# Autodesk Inventor assembly: Field plates
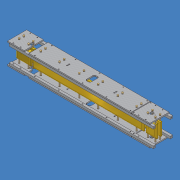
[picture p0: Inventor's stored thumbnail of the model, 180x180]
Saved by Autodesk Inventor 2011 (Build 150239000, 239)
## iProperties
Created: 2005-07-04
Part Number: Field plates
Document SubType Name: Assembly
Designer: jony
Author: jony
## Documents named in this file (5)
- C:\Users\Joe\Inventor\EDM Beamline 2010\EDM Beamline\Field plates\Field plates.iam
- C:\Users\Joe\Inventor\EDM Beamline 2010\EDM Beamline\Field plates\Plate support assembly.iam
- C:\Users\Joe\Inventor\EDM Beamline 2010\EDM Beamline\Field plates\Lower guard assembly.iam
- C:\Users\Joe\Inventor\EDM Beamline 2010\EDM Beamline\Field plates\Upper guard assembly.iam
- C:\Users\Joe\Inventor\EDM Beamline 2010\EDM Beamline\Field plates\C plate assembly.iam
## Components (8 placed, 4 different names)
1. Plate support assembly:1 [sub-assembly] — Mate:1, Mate:2, Mate:3, Mate:4, Mate:7, Mate:8, Mate:9, Mate:10, Mate:11, Mate:12, Mate:13, Mate:14, Mate:15, Mate:16, Mate:17, Mate:18, Mate:19, Mate:20, Mate:21
2. Plate support assembly:2 [sub-assembly] — Mate:5, Mate:6, Mate:15
3. Lower guard assembly:1 [sub-assembly] — Mate:1, Mate:2, Mate:5, Mate:6, Mate:16
4. Lower guard assembly:2 [sub-assembly] — Mate:3, Mate:4, Mate:17
5. Upper guard assembly:1 [sub-assembly] — Mate:7, Mate:8, Mate:18
6. Upper guard assembly:2 [sub-assembly] — Mate:9, Mate:10, Mate:19
7. C plate assembly:1 [sub-assembly] — Mate:11, Mate:12, Mate:20
8. C plate assembly:2 [sub-assembly] — Mate:13, Mate:14, Mate:21
## Relationships (21: Mate 21)
- Mate:1: Plate support assembly:1 ↔ Lower guard assembly:1
- Mate:2: Plate support assembly:1 ↔ Lower guard assembly:1
- Mate:3: Plate support assembly:1 ↔ Lower guard assembly:2
- Mate:4: Plate support assembly:1 ↔ Lower guard assembly:2
- Mate:5: Plate support assembly:2 ↔ Lower guard assembly:1
- Mate:6: Plate support assembly:2 ↔ Lower guard assembly:1
- Mate:7: Plate support assembly:1 ↔ Upper guard assembly:1
- Mate:8: Plate support assembly:1 ↔ Upper guard assembly:1
- Mate:9: Plate support assembly:1 ↔ Upper guard assembly:2
- Mate:10: Plate support assembly:1 ↔ Upper guard assembly:2
- Mate:11: Plate support assembly:1 ↔ C plate assembly:1
- Mate:12: Plate support assembly:1 ↔ C plate assembly:1
- Mate:13: Plate support assembly:1 ↔ C plate assembly:2
- Mate:14: Plate support assembly:1 ↔ C plate assembly:2
- Mate:15 (77.1144 mm): Plate support assembly:1 ↔ Plate support assembly:2
- Mate:16 (38.5572 mm): Plate support assembly:1 ↔ Lower guard assembly:1
- Mate:17 (38.5572 mm): Plate support assembly:1 ↔ Lower guard assembly:2
- Mate:18 (38.5572 mm): Plate support assembly:1 ↔ Upper guard assembly:1
- Mate:19 (38.5572 mm): Plate support assembly:1 ↔ Upper guard assembly:2
- Mate:20 (38.5572 mm): Plate support assembly:1 ↔ C plate assembly:1
- Mate:21 (38.5572 mm): Plate support assembly:1 ↔ C plate assembly:2
